# Autodesk Inventor assembly: Assembly1
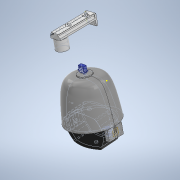
[picture p0: Inventor's stored thumbnail of the model, 180x180]
Saved by Autodesk Inventor 2021.1 (Build 251245010, 245A)
## iProperties
Created: 2023-07-02
Part Number: Assembly1
Document SubType Name: Assembly
Designer: Drake
Author: Drake
## Documents named in this file (6)
- C:\bkp\FYPDESIGN1\Assembly1.iam
- C:\bkp\FYPDESIGN1\TopBracket.ipt
- C:\bkp\FYPDESIGN1\EnclosingRevolver.ipt
- C:\bkp\FYPDESIGN1\CameraHolder2.ipt
- C:\bkp\FYPDESIGN1\SG90_Model_B.ipt
- C:\bkp\FYPDESIGN1\sg90CustomArm.ipt
## Components (6 placed, 5 different names)
1. TopBracket:1
2. EnclosingRevolver:1 — Mate:3, Mate:7, Insert:2
3. CameraHolder2:1 — Mate:3, Mate:5, Mate:6, Insert:1
4. SG90_Model_B:1 — Mate:5, Mate:6, Insert:1, Rotation:1
5. sg90CustomArm:1 — Mate:7, Rotation:1
6. SG90_Model_B:2 — Insert:2
## Relationships (7: Mate 4, Insert 2, RelateRotation 1)
- Mate:3: EnclosingRevolver:1 ↔ CameraHolder2:1
- Mate:5: CameraHolder2:1 ↔ SG90_Model_B:1
- Mate:6: CameraHolder2:1 ↔ SG90_Model_B:1
- Insert:1: CameraHolder2:1 ↔ SG90_Model_B:1
- Mate:7: EnclosingRevolver:1 ↔ sg90CustomArm:1
- Rotation:1 [RelateRotation] (1 ul): SG90_Model_B:1 ↔ sg90CustomArm:1
- Insert:2 (-3.6068 mm): EnclosingRevolver:1 ↔ SG90_Model_B:2
